# Autodesk Inventor assembly: 32 spocket with hub_MIR
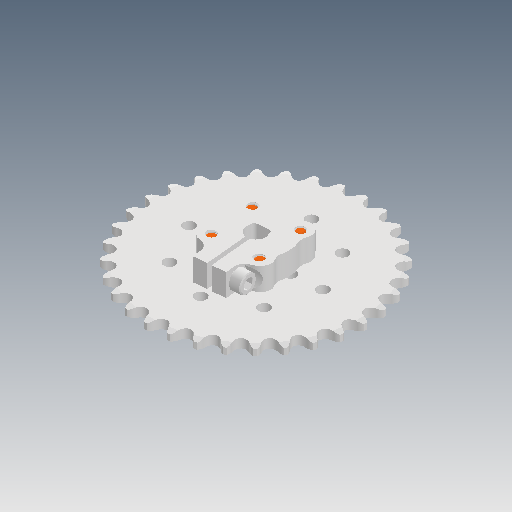
[picture p0: Inventor's stored thumbnail of the model, 512x512]
Saved by Autodesk Inventor 2020 (Build 240168000, 168)
## iProperties
Created: 2019-09-29
Part Number: 32 spocket with hub_MIR
Document SubType Name: Assembly
Designer: ball
Author: ball
## Documents named in this file (4)
- C:\FTC\FTC8863CAD\2019 Robot\Mecanum Drive Train\32 spocket with hub_MIR.iam
- C:\FTC\FTC8863CAD\Actobotics\545 parts\545618 assembly_MIR.ipt
- C:\FTC\FTC8863CAD\Actobotics\615 parts\615114_MIR.ipt
- C:\FTC\FTC8863CAD\Actobotics\632 parts\632110_MIR.ipt
## Components (6 placed, 3 different names)
1. 545618 assembly_MIR:1 — Mate:3, Mate:2, Mate:1, Mate:4, Mate:6
2. 615114_MIR:1 — Mate:3, Mate:2, Mate:1, Mate:5, Mate:7, Mate:11, Mate:8, Mate:10, Mate:9
3. 632110_MIR:1 — Mate:5, Mate:4
4. 632110_MIR:2 — Mate:7, Mate:6
5. 632110_MIR:3 — Mate:11, Mate:8
6. 632110_MIR:4 — Mate:10, Mate:9
## Relationships (11: Mate 11)
- Mate:3: 545618 assembly_MIR:1 ↔ 615114_MIR:1
- Mate:2: 545618 assembly_MIR:1 ↔ 615114_MIR:1
- Mate:1: 545618 assembly_MIR:1 ↔ 615114_MIR:1
- Mate:5: 615114_MIR:1 ↔ 632110_MIR:1
- Mate:4: 545618 assembly_MIR:1 ↔ 632110_MIR:1
- Mate:7: 615114_MIR:1 ↔ 632110_MIR:2
- Mate:6: 545618 assembly_MIR:1 ↔ 632110_MIR:2
- Mate:11: 615114_MIR:1 ↔ 632110_MIR:3
- Mate:8: 615114_MIR:1 ↔ 632110_MIR:3
- Mate:10: 615114_MIR:1 ↔ 632110_MIR:4
- Mate:9: 615114_MIR:1 ↔ 632110_MIR:4
